# Autodesk Inventor assembly: DarthJefkeAssembly
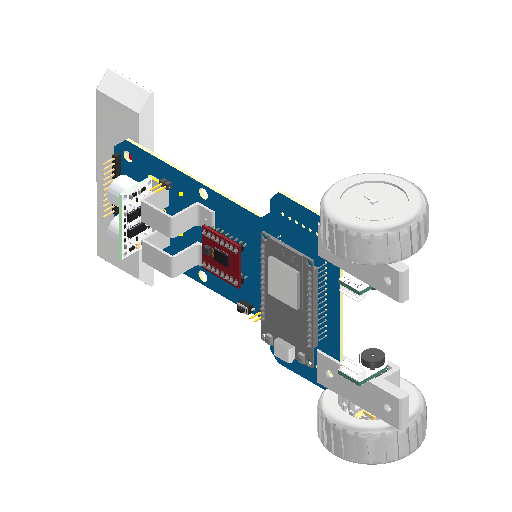
[picture p0: Inventor's stored thumbnail of the model, 512x512]
Saved by Autodesk Inventor 2026.1 (Build 301233020, 233B)
## iProperties
Created: 2026-04-23
Part Number: DarthJefkeAssembly
Document SubType Name: Assembly
Designer: YannickBrusselmans
Author: YannickBrusselmans
## Documents named in this file (12)
- C:\Mac\Home\Documents\ua\Alle files DarthJefke\InventorFiles\DarthJefkeAssembly.iam
- C:\Mac\Home\Documents\ua\Alle files DarthJefke\InventorFiles\esp32.ipt
- C:\Mac\Home\Documents\ua\Alle files DarthJefke\InventorFiles\Motor Mount.ipt
- C:\Mac\Home\Documents\ua\Alle files DarthJefke\InventorFiles\PCB.iam
- C:\Mac\Home\Documents\ua\Alle files DarthJefke\InventorFiles\QTR-8A_TOP.iam
- C:\Mac\Home\Documents\ua\Alle files DarthJefke\InventorFiles\N20 Mini Micro Metall Gear.ipt
- C:\Mac\Home\Documents\ua\Alle files DarthJefke\InventorFiles\tinker.ipt
- C:\Mac\Home\Documents\ua\Alle files DarthJefke\InventorFiles\rcw-0001.ipt
- C:\Mac\Home\Documents\ua\Alle files DarthJefke\InventorFiles\Wiel.ipt
- C:\Mac\Home\Documents\ua\Alle files DarthJefke\InventorFiles\IR-housing.ipt
- C:\Mac\Home\Documents\ua\Alle files DarthJefke\InventorFiles\Batterijbevestiging.ipt
- C:\Mac\Home\Documents\ua\Alle files DarthJefke\InventorFiles\Components_model_Ball_caster_DFrobot.ipt
## Components (14 placed, 11 different names)
1. esp32:1 — Mate:2
2. Motor Mount:1 — Rotational:1, Rigid:1, Rigid:2
3. PCB:1 [sub-assembly] — Mate:2, Cylindrical:1, Rotational:1, Cylindrical:4, Rigid:3, Mate:3, Mate:4, Mate:5, Mate:6
4. QTR-8A_TOP:1 [sub-assembly] — Cylindrical:1
5. N20 Mini Micro Metall Gear:1 — Rigid:1, Rigid:4
6. N20 Mini Micro Metall Gear:2 — Rigid:2, Rigid:5
7. tinker:1 — Cylindrical:4
8. rcw-0001:1 — Rigid:3
9. Wiel:1 — Rigid:4
10. Wiel:2 — Rigid:5
11. IR-housing:1 — Mate:3
12. Batterijbevestiging:1 — Mate:4
13. Batterijbevestiging:2 — Mate:5
14. Components_model_Ball_caster_DFrobot:1 — Mate:6
## Relationships (13: Mate 5, WeldJoint 5, CylindricalJoint 2, RevoluteJoint 1)
- Mate:2: esp32:1 ↔ PCB:1
- Cylindrical:1: PCB:1 ↔ QTR-8A_TOP:1
- Rotational:1 [RevoluteJoint]: Motor Mount:1 ↔ PCB:1
- Rigid:1 [WeldJoint]: Motor Mount:1 ↔ N20 Mini Micro Metall Gear:1
- Rigid:2 [WeldJoint]: Motor Mount:1 ↔ N20 Mini Micro Metall Gear:2
- Cylindrical:4: PCB:1 ↔ tinker:1
- Rigid:3 [WeldJoint]: PCB:1 ↔ rcw-0001:1
- Rigid:4 [WeldJoint]: N20 Mini Micro Metall Gear:1 ↔ Wiel:1
- Rigid:5 [WeldJoint]: N20 Mini Micro Metall Gear:2 ↔ Wiel:2
- Mate:3: PCB:1 ↔ IR-housing:1
- Mate:4: PCB:1 ↔ Batterijbevestiging:1
- Mate:5: PCB:1 ↔ Batterijbevestiging:2
- Mate:6: PCB:1 ↔ Components_model_Ball_caster_DFrobot:1
